# Autodesk Inventor assembly: Assemlby_TIRFImager_v0
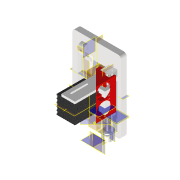
[picture p0: Inventor's stored thumbnail of the model, 180x180]
Saved by Autodesk Inventor 2022 (Build 260153000, 153)
## iProperties
Created: 2022-05-21
Part Number: Assemlby_TIRFImager_v0
Document SubType Name: Assembly
Designer: diederichbenedict
Author: diederichbenedict
## Documents named in this file (8)
- C:\Users\diederichbenedict\Dropbox\Dokumente\Promotion\PROJECTS\TIRFImager\INVENTOR\Assemlby_TIRFImager_v0.iam
- C:\Users\diederichbenedict\Dropbox\Dokumente\Promotion\PROJECTS\TIRFImager\INVENTOR\TIRFImager_base_v0.ipt
- C:\Users\diederichbenedict\Dropbox\Dokumente\Promotion\PROJECTS\TIRFImager\INVENTOR\00_chipnano_waveguide_slidsize.ipt
- C:\Users\diederichbenedict\Dropbox\Dokumente\Promotion\PROJECTS\TIRFImager\INVENTOR\00_LASER_640nm.ipt
- C:\Users\diederichbenedict\Dropbox\Dokumente\Promotion\PROJECTS\TIRFImager\INVENTOR\00_KES400.iam
- C:\Users\diederichbenedict\Dropbox\Dokumente\Promotion\PROJECTS\TIRFImager\INVENTOR\tmp.iam
- C:\Users\diederichbenedict\Dropbox\Dokumente\Promotion\PROJECTS\TIRFImager\INVENTOR\30_XYTabel_Aliexpress_cellSTORM_chiptray_clamp.ipt
- C:\Users\diederichbenedict\Dropbox\Dokumente\Promotion\PROJECTS\TIRFImager\INVENTOR\TIRFImager_Laserbase_v1.ipt
## Components (8 placed, 7 different names)
1. TIRFImager_base_v0:1 — Passend:1, Fluchtend:1, Fluchtend:2, Passend:3, Fluchtend:3, Winkel:3, Fluchtend:6, Einfügen:1, Einfügen:2
2. 00_chipnano_waveguide_slidsize:1 — Passend:1, Fluchtend:1, Fluchtend:2
3. 00_KES400:1 [sub-assembly] — Fluchtend:3, Winkel:3, Passend:6, Passend:7
4. tmp:1 [sub-assembly] — Passend:3, Fluchtend:6
5. 30_XYTabel_Aliexpress_cellSTORM_chiptray_clamp:1 — Einfügen:1
6. 30_XYTabel_Aliexpress_cellSTORM_chiptray_clamp:2 — Einfügen:2
7. TIRFImager_Laserbase_v1:1 — Passend:6, Fluchtend:7
8. 00_LASER_640nm:1 — Passend:7, Fluchtend:7
## Relationships (13: Mate 5, Flush 5, Insert 2, Angle 1)
- Passend:1 [Mate]: TIRFImager_base_v0:1 ↔ 00_chipnano_waveguide_slidsize:1
- Fluchtend:1 [Flush] (1 mm): TIRFImager_base_v0:1 ↔ 00_chipnano_waveguide_slidsize:1
- Fluchtend:2 [Flush] (10 mm): TIRFImager_base_v0:1 ↔ 00_chipnano_waveguide_slidsize:1
- [Mate]: 00_chipnano_waveguide_slidsize:1 ↔ 00_KES400:1
- Passend:3 [Mate]: TIRFImager_base_v0:1 ↔ tmp:1
- Fluchtend:3 [Flush] (3 mm): TIRFImager_base_v0:1 ↔ 00_KES400:1
- Winkel:3 [Angle] (0 deg): TIRFImager_base_v0:1 ↔ 00_KES400:1
- Fluchtend:6 [Flush]: TIRFImager_base_v0:1 ↔ tmp:1
- Einfügen:1 [Insert]: TIRFImager_base_v0:1 ↔ 30_XYTabel_Aliexpress_cellSTORM_chiptray_clamp:1
- Einfügen:2 [Insert]: TIRFImager_base_v0:1 ↔ 30_XYTabel_Aliexpress_cellSTORM_chiptray_clamp:2
- Passend:6 [Mate]: 00_KES400:1 ↔ TIRFImager_Laserbase_v1:1
- Passend:7 [Mate]: 00_KES400:1 ↔ 00_LASER_640nm:1
- Fluchtend:7 [Flush] (-8 mm): TIRFImager_Laserbase_v1:1 ↔ 00_LASER_640nm:1
